# Autodesk Inventor assembly: DoubleCross_Bar_printasm
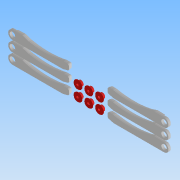
[picture p0: Inventor's stored thumbnail of the model, 180x180]
Saved by Autodesk Inventor 2021 (Build 250183000, 183)
## iProperties
Created: 2021-02-18
Part Number: DoubleCross_Bar_printasm
Document SubType Name: Assembly
Designer: kumagai
Author: kumagai
## Documents named in this file (4)
- Z:\Develop\CAD\PlaRails\DoubleCross\DoubleCross_Bar_printasm.iam
- Z:\Develop\CAD\PlaRails\DoubleCross\DoubleCrossBar.ipt
- Z:\Develop\CAD\PlaRails\DoubleCross\DoubleCrossBar_MIR.ipt
- Z:\Develop\CAD\PlaRails\DoubleCross\DoubleCrossBarPin.ipt
## Components (12 placed, 3 different names)
1. DoubleCrossBar_MIR:1 — フラッシュ:3, メイト:3, フラッシュ:5, フラッシュ:7
2. DoubleCrossBar:1 — フラッシュ:3, メイト:3, フラッシュ:7, フラッシュ:8
3. DoubleCrossBar_MIR:2
4. DoubleCrossBar:2
5. DoubleCrossBar_MIR:3
6. DoubleCrossBar:3
7. DoubleCrossBarPin:1 — フラッシュ:5, フラッシュ:6, フラッシュ:8
8. DoubleCrossBarPin:2
9. DoubleCrossBarPin:3
10. DoubleCrossBarPin:4
11. DoubleCrossBarPin:5
12. DoubleCrossBarPin:6
## Component patterns: (3 elements, first: DoubleCrossBar_MIR:1 + DoubleCrossBar:1), (6 elements, first: DoubleCrossBarPin:1)
## Relationships (6: Flush 5, Mate 1)
- フラッシュ:3 [Flush]: DoubleCrossBar_MIR:1 ↔ DoubleCrossBar:1
- メイト:3 [Mate] (36 mm): DoubleCrossBar_MIR:1 ↔ DoubleCrossBar:1
- フラッシュ:5 [Flush] (4 mm): DoubleCrossBar_MIR:1 ↔ DoubleCrossBarPin:1
- フラッシュ:6 [Flush]: DoubleCrossBarPin:1
- フラッシュ:7 [Flush]: DoubleCrossBar_MIR:1 ↔ DoubleCrossBar:1
- フラッシュ:8 [Flush]: DoubleCrossBar:1 ↔ DoubleCrossBarPin:1
